# Autodesk Inventor assembly: soporte_servo
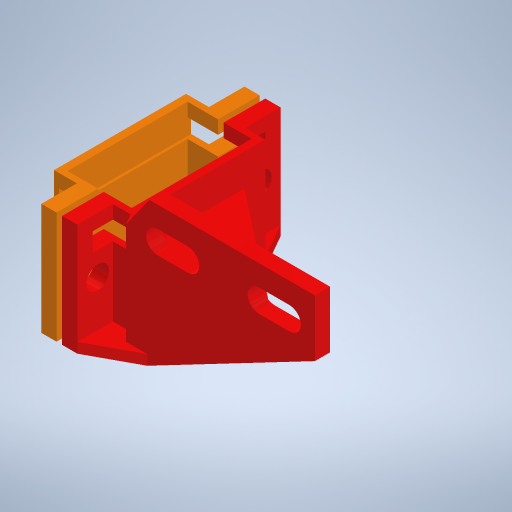
[picture p0: Inventor's stored thumbnail of the model, 512x512]
Saved by Autodesk Inventor 2024.3 (Build 283343000, 343)
## iProperties
Created: 2024-09-30
Part Number: soporte_servo
Document SubType Name: Assembly
Designer: User
Author: User
## Documents named in this file (3)
- C:\Users\User\Documents\Universidad Octavo Semestre\Robotica Industrial\matlab\SCARA\mariana_scara_final\mariana_scara_final\soporte_servo.iam
- C:\Users\User\Documents\Universidad Octavo Semestre\Robotica Industrial\matlab\SCARA\mariana_scara_final\mariana_scara_final\soporte-motor.ipt
- C:\Users\User\Documents\Universidad Octavo Semestre\Robotica Industrial\matlab\SCARA\mariana_scara_final\mariana_scara_final\soprte_motor.ipt
## Components (2 placed, 2 different names)
1. soporte-motor:1 — Mate:1, Flush:1, Flush:2
2. soprte_motor:1 — Mate:1, Flush:1, Flush:2
## Relationships (3: Flush 2, Mate 1)
- Mate:1 (1.1 mm): soporte-motor:1 ↔ soprte_motor:1
- Flush:1: soporte-motor:1 ↔ soprte_motor:1
- Flush:2: soporte-motor:1 ↔ soprte_motor:1
